# Autodesk Inventor assembly: Arm for Gen 2
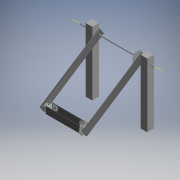
[picture p0: Inventor's stored thumbnail of the model, 180x180]
Saved by Autodesk Inventor 2019 (Build 230136000, 136)
## iProperties
Part Number: Arm for Gen 2
Document SubType Name: Assembly
Designer: Delta
Author: Delta
## Documents named in this file (9)
- C:\Robotics\2019-20_CAD\Collection\Arm for Gen 2.iam
- C:\Robotics\2019-20_CAD\Collection\30x30 pillars.ipt
- C:\Robotics\2019-20_CAD\Collection\12 Inch Hex Axle.ipt
- C:\Robotics\COTSParts\Sprockets - AndyMark\615106.ipt
- C:\Robotics\2019-20_CAD\Collection\bar arms.ipt
- C:\Robotics\2019-20_CAD\Collection\Claw holding bars.ipt
- C:\Robotics\COTSParts\Tetrix\39270_txm-insidecconnectors.ipt
- C:\Robotics\COTSParts\Actobotics\545 parts\545364 assembly.ipt
- C:\Robotics\COTSParts\Actobotics\545 parts\545456PatternAdapter.77in.625in.ipt
## Components (14 placed, 8 different names)
1. 30x30 pillars:1 — Mate:2, Flush:2, Mate:11, Mate:21
2. 30x30 pillars:2 — Mate:3, Flush:2, Mate:11, Angle:1, Flush:6
3. 12 Inch Hex Axle:1 — Mate:2, Mate:3, Mate:5, Mate:6, Mate:8, Flush:6
4. 615106:1 — Mate:5, Mate:51
5. bar arms:1 — Mate:6, Flush:5, Mate:21, Mate:41, Mate:50
6. bar arms:2 — Mate:8, Flush:5, Mate:45, Mate:51
7. Claw holding bars:1 — Angle:1, Mate:22, Mate:23, Mate:24, Mate:25, Mate:26, Mate:27
8. 615106:2 — Mate:46, Mate:47, Mate:48, Mate:49
9. 39270_txm-insidecconnectors:1 — Mate:25, Mate:26, Mate:27, Mate:31, Mate:32
10. 39270_txm-insidecconnectors:2 — Mate:22, Mate:23, Mate:24, Mate:29, Mate:42, Mate:43
11. 545364 assembly:1 — Mate:33, Mate:35, Mate:45, Mate:47
12. 545364 assembly:2 — Mate:37, Mate:38, Mate:39, Mate:41, Mate:50
13. 545456PatternAdapter.77in.625in:1 — Mate:31, Mate:32, Mate:33, Mate:35, Mate:46, Mate:48, Mate:49
14. 545456PatternAdapter.77in.625in:2 — Mate:29, Mate:37, Mate:38, Mate:39, Mate:42, Mate:43
## Relationships (35: Mate 31, Flush 3, Angle 1)
- Mate:2: 30x30 pillars:1 ↔ 12 Inch Hex Axle:1
- Mate:3: 30x30 pillars:2 ↔ 12 Inch Hex Axle:1
- Flush:2: 30x30 pillars:1 ↔ 30x30 pillars:2
- Mate:5: 12 Inch Hex Axle:1 ↔ 615106:1
- Mate:6: 12 Inch Hex Axle:1 ↔ bar arms:1
- Mate:8: 12 Inch Hex Axle:1 ↔ bar arms:2
- Flush:5: bar arms:1 ↔ bar arms:2
- Mate:11 (230.632 mm): 30x30 pillars:1 ↔ 30x30 pillars:2
- Angle:1 (270 deg): 30x30 pillars:2 ↔ Claw holding bars:1
- Mate:21 (11.43 mm): 30x30 pillars:1 ↔ bar arms:1
- Mate:22: Claw holding bars:1 ↔ 39270_txm-insidecconnectors:2
- Mate:23: Claw holding bars:1 ↔ 39270_txm-insidecconnectors:2
- Mate:24: Claw holding bars:1 ↔ 39270_txm-insidecconnectors:2
- Mate:25: Claw holding bars:1 ↔ 39270_txm-insidecconnectors:1
- Mate:26: Claw holding bars:1 ↔ 39270_txm-insidecconnectors:1
- Mate:27: Claw holding bars:1 ↔ 39270_txm-insidecconnectors:1
- Mate:29: 39270_txm-insidecconnectors:2 ↔ 545456PatternAdapter.77in.625in:2
- Mate:31: 39270_txm-insidecconnectors:1 ↔ 545456PatternAdapter.77in.625in:1
- Mate:32: 39270_txm-insidecconnectors:1 ↔ 545456PatternAdapter.77in.625in:1
- Mate:33: 545364 assembly:1 ↔ 545456PatternAdapter.77in.625in:1
- Mate:35: 545364 assembly:1 ↔ 545456PatternAdapter.77in.625in:1
- Mate:37: 545364 assembly:2 ↔ 545456PatternAdapter.77in.625in:2
- Mate:38: 545364 assembly:2 ↔ 545456PatternAdapter.77in.625in:2
- Mate:39: 545364 assembly:2 ↔ 545456PatternAdapter.77in.625in:2
- Mate:41: bar arms:1 ↔ 545364 assembly:2
- Mate:42: 39270_txm-insidecconnectors:2 ↔ 545456PatternAdapter.77in.625in:2
- Mate:43 (0.0762 mm): 39270_txm-insidecconnectors:2 ↔ 545456PatternAdapter.77in.625in:2
- Mate:45: bar arms:2 ↔ 545364 assembly:1
- Mate:46: 615106:2 ↔ 545456PatternAdapter.77in.625in:1
- Mate:47: 615106:2 ↔ 545364 assembly:1
- Mate:48: 615106:2 ↔ 545456PatternAdapter.77in.625in:1
- Mate:49: 615106:2 ↔ 545456PatternAdapter.77in.625in:1
- Mate:50: bar arms:1 ↔ 545364 assembly:2
- Mate:51 (9.6266 mm): 615106:1 ↔ bar arms:2
- Flush:6 (-19.05 mm): 30x30 pillars:2 ↔ 12 Inch Hex Axle:1
